# Autodesk Inventor assembly: Power_Reality_Assembled
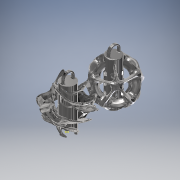
[picture p0: Inventor's stored thumbnail of the model, 180x180]
Saved by Autodesk Inventor 2019 (Build 230136000, 136)
## iProperties
Created: 2019-06-12
Part Number: Power_Reality_Assembled
Document SubType Name: Assembly
Designer: Jorian Bruslind
Author: Jorian Bruslind
## Documents named in this file (3)
- C:\Users\Jorian Bruslind\Documents\GitHub\PersonalProjects\Inventor Projects\Infinity\Power_Reality_Assembled.iam
- C:\Users\Jorian Bruslind\Documents\GitHub\PersonalProjects\Inventor Projects\Infinity\Orb.ipt
- C:\Users\Jorian Bruslind\Documents\GitHub\PersonalProjects\Inventor Projects\Infinity\Waves.ipt
## Components (2 placed, 2 different names)
1. Orb:1 — Flush:1, Mate:1
2. Waves:1 — Flush:1, Mate:1
## Relationships (2: Flush 1, Mate 1)
- Flush:1: Orb:1 ↔ Waves:1
- Mate:1 (12 mm): Orb:1 ↔ Waves:1
